# Autodesk Inventor assembly: Controller_V1
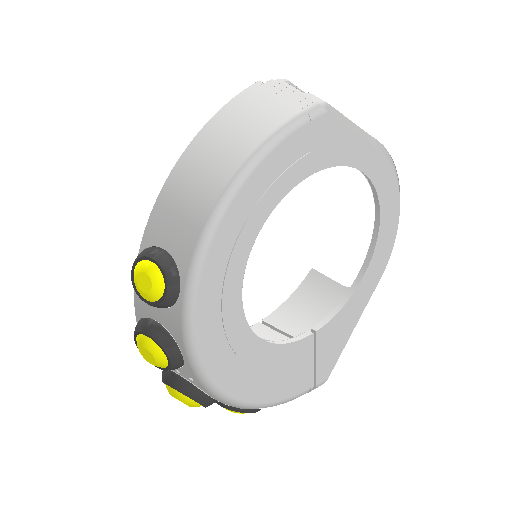
[picture p0: Inventor's stored thumbnail of the model, 512x512]
Saved by Autodesk Inventor 2025.3 (Build 293356030, 356C)
## iProperties
Created: 2025-04-17
Part Number: Controller_V1
Document SubType Name: Assembly
Designer: Andreas
Author: Andreas
## Documents named in this file (7)
- C:\Daten\Temp\AdventureController\cad\Controller_V1.iam
- C:\Daten\Temp\AdventureController\cad\nrf52840.ipt
- C:\Daten\Temp\AdventureController\cad\UpperPartFront.ipt
- C:\Daten\Temp\AdventureController\cad\UperPartBack.ipt
- C:\Daten\Temp\AdventureController\cad\LowerPart.ipt
- C:\Daten\Temp\AdventureController\cad\Nut.ipt
- C:\Daten\Temp\AdventureController\cad\Button_RS_14mm_yellow\Button_RS_14mm_yellow.ipt
## Components (12 placed, 6 different names)
1. UpperPartFront:1 — Insert:1, Mate:1, Flush:1, Flush:2, Flush:3, Tangent:1, Tangent:2, Mate:2, Mate:3, Mate:5, Mate:8
2. nrf52840:1 — Mate:1, Tangent:1, Tangent:2
3. UperPartBack:1 — Mate:2, Mate:3, Mate:5, Mate:6, Flush:4, Angle:1
4. LowerPart:1 — Mate:6, Flush:4, Angle:1
5. Button_RS_14mm_yellow:5 [sub-assembly] — Insert:1, Mate:7
6. Nut:1 — Mate:7, Mate:8
7. Button_RS_14mm_yellow:6 [sub-assembly]
8. Nut:2
9. Button_RS_14mm_yellow:7 [sub-assembly]
10. Nut:3
11. Button_RS_14mm_yellow:8 [sub-assembly]
12. Nut:4
## Component patterns: (4 elements, first: Button_RS_14mm_yellow:5 + Nut:1)
## Relationships (15: Mate 7, Flush 4, Tangent 2, Insert 1, Angle 1)
- Insert:1: UpperPartFront:1 ↔ Button_RS_14mm_yellow:5
- Mate:1: UpperPartFront:1 ↔ nrf52840:1
- Flush:1: UpperPartFront:1
- Flush:2: UpperPartFront:1
- Flush:3: UpperPartFront:1
- Tangent:1 (-6 mm): UpperPartFront:1 ↔ nrf52840:1
- Tangent:2 (-2 mm): UpperPartFront:1 ↔ nrf52840:1
- Mate:2: UpperPartFront:1 ↔ UperPartBack:1
- Mate:3: UpperPartFront:1 ↔ UperPartBack:1
- Mate:5: UpperPartFront:1 ↔ UperPartBack:1
- Mate:6: UperPartBack:1 ↔ LowerPart:1
- Flush:4: UperPartBack:1 ↔ LowerPart:1
- Angle:1 (180 deg): UperPartBack:1 ↔ LowerPart:1
- Mate:7: Button_RS_14mm_yellow:5 ↔ Nut:1
- Mate:8: UpperPartFront:1 ↔ Nut:1
